# Autodesk Inventor assembly: sestava tělo estonsko s plechem otočené motory
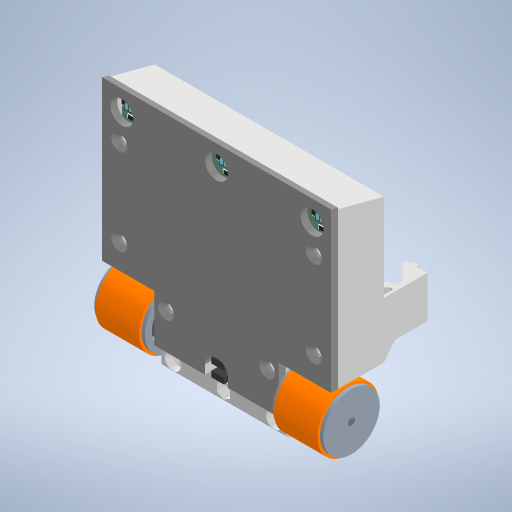
[picture p0: Inventor's stored thumbnail of the model, 512x512]
Saved by Autodesk Inventor 2024 (Build 280153000, 153)
## iProperties
Created: 2023-11-12
Part Number: sestava tělo estonsko s plechem otočené motory
Document SubType Name: Assembly
Designer: 42060
Author: 42060
## Documents named in this file (8)
- C:\Users\42060\Desktop\ŠKOLA\Mini sumo\RoboCop\- 3D -\wip\Tělo s plechem\sestava tělo estonsko s plechem otočené motory.iam
- C:\Users\42060\Desktop\ŠKOLA\Mini sumo\RoboCop\- 3D -\wip\Tělo s plechem\motor_C_clamp_nutt_motor_otoceny.ipt
- C:\Users\42060\Desktop\ŠKOLA\Mini sumo\RoboCop\- 3D -\wip\Tělo s plechem\tělo estonsko s plechem otočené motory.ipt
- C:\Users\42060\Desktop\ŠKOLA\Mini sumo\RoboCop\- 3D -\el._parts\GA12-N20_Motor.ipt
- C:\Users\42060\Desktop\ŠKOLA\Mini sumo\RoboCop\- 3D -\mech._parts\plech.ipt
- C:\Users\42060\Desktop\ŠKOLA\Mini sumo\RoboCop\- 3D -\mech._parts\wheel+silicon.ipt
- C:\Users\42060\Desktop\ŠKOLA\Mini sumo\RoboCop\- 3D -\el._parts\qre_module.ipt
- C:\Users\42060\Desktop\ŠKOLA\Mini sumo\RoboCop\- 3D -\el._parts\sumec_smd.iam
## Components (10 placed, 7 different names)
1. motor_C_clamp_nutt_motor_otoceny:1 — Tuhé:1
2. tělo estonsko s plechem otočené motory:1 — Tuhé:1, Tuhé:2, Proti sobě:1, Proti sobě:2, Stejný směr:1, Proti sobě:3, Stejný směr:2, Proti sobě:4, Tuhé:3, Tuhé:4, Tuhé:5
3. motor_C_clamp_nutt_motor_otoceny:2 — Tuhé:2
4. GA12-N20_Motor:1 — Proti sobě:1, Proti sobě:2, Stejný směr:1, Rotační:1
5. GA12-N20_Motor:2 — Proti sobě:3, Stejný směr:2, Proti sobě:4, Rotační:2
6. plech:1 — Tuhé:3
7. wheel+silicon:1 — Rotační:1
8. wheel+silicon:2 — Rotační:2
9. qre_module:1 — Tuhé:4
10. sumec_smd:1 [sub-assembly] — Tuhé:5
## Relationships (13: WeldJoint 5, Mate 4, Flush 2, RevoluteJoint 2)
- Tuhé:1 [WeldJoint] (-1 mm): motor_C_clamp_nutt_motor_otoceny:1 ↔ tělo estonsko s plechem otočené motory:1
- Tuhé:2 [WeldJoint] (-1 mm): tělo estonsko s plechem otočené motory:1 ↔ motor_C_clamp_nutt_motor_otoceny:2
- Proti sobě:1 [Mate]: tělo estonsko s plechem otočené motory:1 ↔ GA12-N20_Motor:1
- Proti sobě:2 [Mate] (0.1 mm): tělo estonsko s plechem otočené motory:1 ↔ GA12-N20_Motor:1
- Stejný směr:1 [Flush]: tělo estonsko s plechem otočené motory:1 ↔ GA12-N20_Motor:1
- Proti sobě:3 [Mate]: tělo estonsko s plechem otočené motory:1 ↔ GA12-N20_Motor:2
- Stejný směr:2 [Flush]: tělo estonsko s plechem otočené motory:1 ↔ GA12-N20_Motor:2
- Proti sobě:4 [Mate] (0.1 mm): tělo estonsko s plechem otočené motory:1 ↔ GA12-N20_Motor:2
- Tuhé:3 [WeldJoint]: tělo estonsko s plechem otočené motory:1 ↔ plech:1
- Rotační:1 [RevoluteJoint]: GA12-N20_Motor:1 ↔ wheel+silicon:1
- Rotační:2 [RevoluteJoint]: GA12-N20_Motor:2 ↔ wheel+silicon:2
- Tuhé:4 [WeldJoint]: tělo estonsko s plechem otočené motory:1 ↔ qre_module:1
- Tuhé:5 [WeldJoint]: tělo estonsko s plechem otočené motory:1 ↔ sumec_smd:1
